# Autodesk Inventor assembly: frame
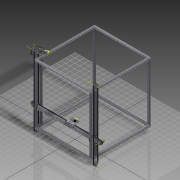
[picture p0: Inventor's stored thumbnail of the model, 180x180]
Saved by Autodesk Inventor 2013 (Build 170138000, 138)
## iProperties
Created: 2013-09-09
Part Number: frame
Document SubType Name: Assembly
Designer: Ian
Mass: 20029.5 g
Surface Area: 72396 cm^2
Volume: 16186.8 cm^3
Density: 1.2374 g/cm^3
Author: Ian
## Documents named in this file (8)
- C:\Users\Ian\Documents\Inventor\xyPartStorage\frame.iam
- C:\Users\Ian\Documents\Inventor\xyPartStorage\frame\Design Accelerator\Synchronous Belts Transmission1.iam
- C:\Users\Ian\Documents\Inventor\xyPartStorage\loader\xyArmature.iam
- C:\Users\Ian\Documents\Inventor\xyPartStorage\loader\sub-frame.iam
- C:\Users\Ian\Documents\Inventor\xyPartStorage\frame\Design Accelerator\Synchronous Belts Transmission2.iam
- C:\Users\Ian\Documents\Inventor\xyPartStorage\frame\Design Accelerator\Synchronous Belts Transmission4.iam
- C:\Users\Ian\Documents\Inventor\xyPartStorage\loader\y_motor_mount.ipt
- C:\Users\Ian\Documents\Inventor\xyPartStorage\stepper\NEMA_17.ipt
## Components (8 placed, 5 different names)
1. sub-frame:1 [sub-assembly] — Mate:55, Mate:61, Flush:4, Mate:5
2. Synchronous Belts Transmission:1 [sub-assembly] — Flush:1, Flush:3
3. xyArmature:1 [sub-assembly] — Flush:1, Flush:2, Mate:58
4. Synchronous Belts Transmission:2 [sub-assembly] — Flush:2, Mate:53, Mate:54, Mate:55, Mate:56, Mate:57, Mate:59, Mate:60
5. Synchronous Belts Transmission:3 [sub-assembly] — Mate:56, Mate:57, Mate:58
6. Synchronous Belts Transmission:4 [sub-assembly] — Mate:59, Mate:60, Mate:61, Mate:62, Mate:63
7. y_motor_mount:1 — Mate:62, Flush:4, Mate:5, Mate:64, Mate:65
8. NEMA_17:1 — Mate:63, Mate:64, Mate:65
## Relationships (29: Mate 25, Flush 4)
- [Mate]: sub-frame:1 ↔ xyArmature:1
- [Mate]: sub-frame:1 ↔ xyArmature:1
- [Mate]: sub-frame:1 ↔ xyArmature:1
- [Mate]: sub-frame:1 ↔ xyArmature:1
- [Mate]: sub-frame:1 ↔ xyArmature:1
- [Mate]: sub-frame:1 ↔ xyArmature:1
- [Mate]: sub-frame:1 ↔ xyArmature:1
- [Mate]: sub-frame:1 ↔ xyArmature:1
- [Mate]: sub-frame:1 ↔ xyArmature:1
- [Mate]: Synchronous Belts Transmission:1 ↔ xyArmature:1
- [Mate] (-35.7124 mm): Synchronous Belts Transmission:1 ↔ xyArmature:1
- Flush:1 (7.62 mm): Synchronous Belts Transmission:1 ↔ xyArmature:1
- Flush:2 (12.7 mm): xyArmature:1 ↔ Synchronous Belts Transmission:2
- Flush:3 (-9.525 mm): Synchronous Belts Transmission:1
- Mate:53: Synchronous Belts Transmission:2
- Mate:54: Synchronous Belts Transmission:2
- Mate:55 (57.15 mm): sub-frame:1 ↔ Synchronous Belts Transmission:2
- Mate:56: Synchronous Belts Transmission:2 ↔ Synchronous Belts Transmission:3
- Mate:57: Synchronous Belts Transmission:2 ↔ Synchronous Belts Transmission:3
- Mate:58 (-12.7 mm): xyArmature:1 ↔ Synchronous Belts Transmission:3
- Mate:59: Synchronous Belts Transmission:2 ↔ Synchronous Belts Transmission:4
- Mate:60 (6.35 mm): Synchronous Belts Transmission:2 ↔ Synchronous Belts Transmission:4
- Mate:61 (40.5892 mm): sub-frame:1 ↔ Synchronous Belts Transmission:4
- Mate:62: Synchronous Belts Transmission:4 ↔ y_motor_mount:1
- Flush:4: sub-frame:1 ↔ y_motor_mount:1
- Mate:5: sub-frame:1 ↔ y_motor_mount:1
- Mate:63: Synchronous Belts Transmission:4 ↔ NEMA_17:1
- Mate:64: y_motor_mount:1 ↔ NEMA_17:1
- Mate:65: y_motor_mount:1 ↔ NEMA_17:1
